# Autodesk Inventor assembly: kanure
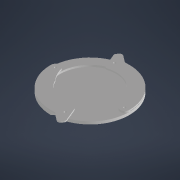
[picture p0: Inventor's stored thumbnail of the model, 180x180]
Saved by Autodesk Inventor 2022 (Build 260153000, 153)
## iProperties
Created: 2023-06-03
Part Number: kanure
Document SubType Name: Assembly
Designer: nyxeon
Author: nyxeon
## Documents named in this file (3)
- C:\Users\nyxeon\Documents\CAD\Inventor\cook\canere\canere.iam
- C:\Users\nyxeon\Documents\CAD\Inventor\cook\canere\canere_01.ipt
- C:\Users\nyxeon\Documents\CAD\Inventor\cook\canere\canere_02.ipt
## Components (3 placed, 2 different names)
1. canere_01:1 — メイト:1, メイト:2, メイト:3, メイト:4
2. canere_02:1 — メイト:1, メイト:2
3. canere_02:2 — メイト:3, メイト:4
## Relationships (4: Mate 4)
- メイト:1 [Mate]: canere_01:1 ↔ canere_02:1
- メイト:2 [Mate] (0.05 mm): canere_01:1 ↔ canere_02:1
- メイト:3 [Mate]: canere_01:1 ↔ canere_02:2
- メイト:4 [Mate] (0.05 mm): canere_01:1 ↔ canere_02:2
